# Autodesk Inventor assembly: DC Motor Assembly
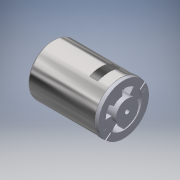
[picture p0: Inventor's stored thumbnail of the model, 180x180]
Saved by Autodesk Inventor 2016 (Build 200138000, 138)
## iProperties
Created: 2015-05-20
Part Number: DC Motor Assembly
Document SubType Name: Assembly
Designer: jonathan
Author: jonathan
## Documents named in this file (3)
- C:\Users\jonathan\Desktop\Motor\DC Motor Assembly.iam
- C:\Users\jonathan\Desktop\Motor\Motor Casing.ipt
- C:\Users\jonathan\Desktop\Motor\Motor Endcap.ipt
## Components (2 placed, 2 different names)
1. Motor Casing:1 — Mate:1, Mate:2
2. Motor Endcap:1 — Mate:1, Mate:2
## Relationships (2: Mate 2)
- Mate:1: Motor Casing:1 ↔ Motor Endcap:1
- Mate:2: Motor Casing:1 ↔ Motor Endcap:1
